# Autodesk Inventor assembly: Test_assembly
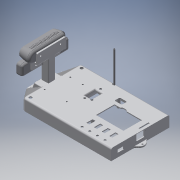
[picture p0: Inventor's stored thumbnail of the model, 180x180]
Saved by Autodesk Inventor 2019 (Build 230136000, 136)
## iProperties
Created: 2020-02-14
Part Number: Test_assembly
Document SubType Name: Assembly
Designer: close
Author: close
## Documents named in this file (11)
- C:\Users\close\Desktop\BARC-ROAR\barc_hardware\Enclosure\V_5\Test_assembly_v5.iam
- C:\Users\close\Desktop\BARC-ROAR\barc_hardware\Enclosure\V_5\Enclosure_v5.ipt
- C:\Users\close\Desktop\BARC-ROAR\barc_hardware\Dependencies\Nvidia Jetson Nano\P3450_P3449_A02_P3448_A02.iam
- C:\Users\close\Desktop\BARC-ROAR\barc_hardware\Dependencies\Splitter Board\SplitterBoard.iam
- C:\Users\close\Desktop\BARC-ROAR\barc_hardware\Dependencies\Arduino\Mega\arduinoMegaDetailed.ipt
- C:\Users\close\Desktop\BARC-ROAR\barc_hardware\Dependencies\Drok Step Down\CN2596-2.iam
- C:\Users\close\Desktop\BARC-ROAR\barc_hardware\Enclosure\V_5\Camera Mount 30mm.ipt
- C:\Users\close\Desktop\BARC-ROAR\barc_hardware\Enclosure\V_5\Dual Camera Mount.ipt
- C:\Users\close\Desktop\BARC-ROAR\barc_hardware\Dependencies\Intel RealSense\D435i\Intel_RealSense_Depth_Camera_D435.iam
- C:\Users\close\Desktop\BARC-ROAR\barc_hardware\Dependencies\Intel RealSense\T265\Intel_RealSense_Tracking_Camera_T265.iam
- C:\Users\close\Desktop\BARC-ROAR\barc_hardware\Enclosure\V_5\Antenna.ipt
## Components (10 placed, 10 different names)
1. Enclosure_v5:1 — Insert:1, Insert:2, Insert:3, Insert:4, Insert:5, Insert:7, Insert:8, Insert:10, Flush:3, Mate:1, Insert:16, Mate:2
2. P3450_P3449_A02_P3448_A02:1 [sub-assembly] — Insert:1, Insert:2
3. SplitterBoard:1 [sub-assembly] — Insert:3, Insert:4
4. arduinoMegaDetailed:1 — Insert:5
5. CN2596-2:1 [sub-assembly] — Insert:7, Insert:8
6. Camera Mount 30mm:1 — Insert:10, Insert:11, Flush:2, Flush:3, Mate:1, Mate:2
7. Dual Camera Mount:1 — Insert:11, Flush:2, Insert:12, Insert:13, Insert:14, Insert:15
8. Intel_RealSense_Depth_Camera_D435:1 [sub-assembly] — Insert:14, Insert:15
9. Intel_RealSense_Tracking_Camera_T265:1 [sub-assembly] — Insert:12, Insert:13
10. Antenna:1 — Insert:16
## Relationships (18: Insert 14, Flush 2, Mate 2)
- Insert:1: Enclosure_v5:1 ↔ P3450_P3449_A02_P3448_A02:1
- Insert:2: Enclosure_v5:1 ↔ P3450_P3449_A02_P3448_A02:1
- Insert:3: Enclosure_v5:1 ↔ SplitterBoard:1
- Insert:4: Enclosure_v5:1 ↔ SplitterBoard:1
- Insert:5: Enclosure_v5:1 ↔ arduinoMegaDetailed:1
- Insert:7: Enclosure_v5:1 ↔ CN2596-2:1
- Insert:8: Enclosure_v5:1 ↔ CN2596-2:1
- Insert:10: Enclosure_v5:1 ↔ Camera Mount 30mm:1
- Insert:11: Camera Mount 30mm:1 ↔ Dual Camera Mount:1
- Flush:2: Camera Mount 30mm:1 ↔ Dual Camera Mount:1
- Insert:12: Dual Camera Mount:1 ↔ Intel_RealSense_Tracking_Camera_T265:1
- Insert:13: Dual Camera Mount:1 ↔ Intel_RealSense_Tracking_Camera_T265:1
- Insert:14: Dual Camera Mount:1 ↔ Intel_RealSense_Depth_Camera_D435:1
- Insert:15: Dual Camera Mount:1 ↔ Intel_RealSense_Depth_Camera_D435:1
- Flush:3 (21 mm): Enclosure_v5:1 ↔ Camera Mount 30mm:1
- Mate:1: Enclosure_v5:1 ↔ Camera Mount 30mm:1
- Insert:16: Enclosure_v5:1 ↔ Antenna:1
- Mate:2: Enclosure_v5:1 ↔ Camera Mount 30mm:1
